# Autodesk Inventor assembly: 3136 1133 82
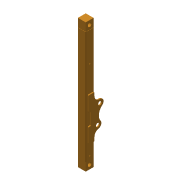
[picture p0: Inventor's stored thumbnail of the model, 180x180]
Saved by Autodesk Inventor 2022 Beta2 (Build 260130000, 130) ContinuousBuild 0
## iProperties
Shininess: 64.0
Length Units: 11269
Angle Units: 11279
Time Units: 11290
Mass Units: 11283
Length Display Precision: 3
Angle Display Precision: 2
Compacted: True
Created: 2003-04-13
Part Number: 3136 1133 82
Document SubType Name: Assembly
Designer: Uffe Bak
Density: 0.0
Volumn: 0.0
Area: 0.0
PropertySet Name: Model Information
Control State: 0
Master: False
Checked Out: False
Author: Uffe Bak
## Documents named in this file (4)
- C:\Autodesk Inventor 2021 Intro Practice Files\BOM\3136 1133 82.iam
- C:\Autodesk Inventor 2021 Intro Practice Files\BOM\3136 1094 48.ipt
- C:\Autodesk Inventor 2021 Intro Practice Files\BOM\3136 1094 44.ipt
- C:\Autodesk Inventor 2021 Intro Practice Files\BOM\3136 1133 83.ipt
## Components (5 placed, 3 different names)
1. 3136 1094 48:1 — Flush:1, Mate:1, Flush:2, Flush:4, Flush:6, Flush:7, Mate:2, Mate:3
2. 3136 1094 44:1 — Flush:1, Flush:2, Flush:3, Flush:4, Flush:5
3. 3136 1094 44:2 — Mate:1, Flush:3, Flush:5
4. 3136 1133 83:1 — Flush:6, Flush:7, Mate:2, Flush:8, Mate:4
5. 3136 1133 83:2 — Mate:3, Flush:8, Mate:4
## Relationships (12: Flush 8, Mate 4)
- Flush:1: 3136 1094 48:1 ↔ 3136 1094 44:1
- Mate:1: 3136 1094 48:1 ↔ 3136 1094 44:2
- Flush:2 (2 mm): 3136 1094 48:1 ↔ 3136 1094 44:1
- Flush:3: 3136 1094 44:1 ↔ 3136 1094 44:2
- Flush:4 (2 mm): 3136 1094 48:1 ↔ 3136 1094 44:1
- Flush:5: 3136 1094 44:1 ↔ 3136 1094 44:2
- Flush:6: 3136 1094 48:1 ↔ 3136 1133 83:1
- Flush:7 (40 mm): 3136 1094 48:1 ↔ 3136 1133 83:1
- Mate:2 (-265.3 mm): 3136 1094 48:1 ↔ 3136 1133 83:1
- Mate:3: 3136 1094 48:1 ↔ 3136 1133 83:2
- Flush:8: 3136 1133 83:1 ↔ 3136 1133 83:2
- Mate:4: 3136 1133 83:1 ↔ 3136 1133 83:2
